# Autodesk Inventor assembly: Assembly1
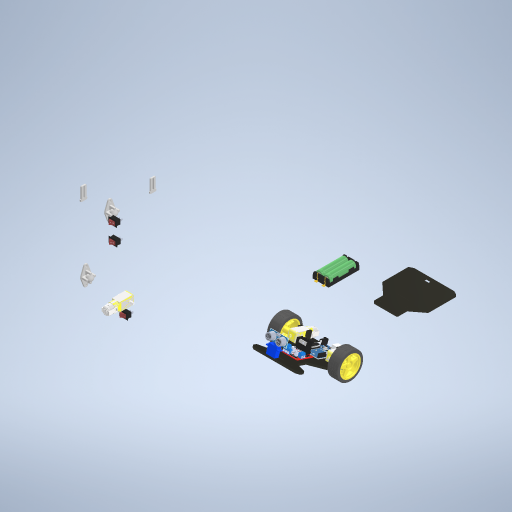
[picture p0: Inventor's stored thumbnail of the model, 512x512]
Saved by Autodesk Inventor 2023 (Build 270158000, 158)
## iProperties
Created: 2023-03-17
Part Number: Assembly1
Document SubType Name: Assembly
Designer: Admins
Author: Admins
## Documents named in this file (15)
- D:\Documents\Researches\Line-Follower-Robot\Assembly1.iam
- D:\Documents\Researches\Line-Follower-Robot\DeTren.ipt
- D:\Documents\Researches\Line-Follower-Robot\KhungDuoi.ipt
- D:\Documents\Researches\Line-Follower-Robot\Parts\Arduino Uno.ipt
- D:\Documents\Researches\Line-Follower-Robot\Parts\Ga motor 1.ipt
- D:\Documents\Researches\Line-Follower-Robot\Parts\HC-SR04.ipt
- D:\Documents\Researches\Line-Follower-Robot\Parts\L298N Stepper Motor Driver (Red).ipt
- D:\Documents\Researches\Line-Follower-Robot\Parts\RockerSwitch.ipt
- D:\Documents\Researches\Line-Follower-Robot\Parts\W420 Ball Caster.ipt
- D:\Documents\Researches\Line-Follower-Robot\Parts\Wheel.ipt
- D:\Documents\Researches\Line-Follower-Robot\Parts\Yellow gear motor.ipt
- D:\Documents\Researches\Line-Follower-Robot\Parts\18650 battery holder.ipt
- D:\Documents\Researches\Line-Follower-Robot\Parts\Yellow gear motor_MIR.ipt
- D:\Documents\Researches\Line-Follower-Robot\Parts\Ga motor 1_MIR.ipt
- D:\Documents\servo-motor-sg90-3.snapshot.3\Servo Motor SG90.ipt
## Components (23 placed, 14 different names)
1. DeTren:1
2. KhungDuoi:1 — Mate:1, Mate:2, Mate:3, Mate:4, Mate:5, Mate:7, Symmetry:1, Mate:12, Flush:1, Mate:15, Flush:2, Mate:17
3. Arduino Uno:1 — Flush:1, Mate:15, Flush:2, Mate:16
4. Ga motor 1:1
5. HC-SR04:1 — Mate:18
6. L298N Stepper Motor Driver (Red):1 — Mate:16
7. RockerSwitch:1
8. W420 Ball Caster:1
9. Wheel:1 — Mate:14
10. Yellow gear motor:1
11. RockerSwitch:2
12. W420 Ball Caster:2
13. Wheel:2 — Mate:13
14. Yellow gear motor:2 — Mate:8, Mate:9, Mate:14
15. 18650 battery holder:1
16. RockerSwitch:3
17. Ga motor 1:2
18. Ga motor 1:3 — Mate:1, Mate:2, Mate:3, Mate:8, Symmetry:1
19. Ga motor 1:4 — Mate:4, Mate:5, Mate:7, Mate:9
20. Yellow gear motor_MIR:1 — Mate:10, Mate:11, Mate:12, Mate:13
21. Ga motor 1_MIR:1 — Mate:10
22. Ga motor 1_MIR:2 — Mate:11
23. Servo Motor SG90:1 — Mate:17, Mate:18
## Relationships (20: Mate 17, Flush 2, Symmetry 1)
- Mate:1: KhungDuoi:1 ↔ Ga motor 1:3
- Mate:2: KhungDuoi:1 ↔ Ga motor 1:3
- Mate:3: KhungDuoi:1 ↔ Ga motor 1:3
- Mate:4: KhungDuoi:1 ↔ Ga motor 1:4
- Mate:5: KhungDuoi:1 ↔ Ga motor 1:4
- Mate:7: KhungDuoi:1 ↔ Ga motor 1:4
- Mate:8: Yellow gear motor:2 ↔ Ga motor 1:3
- Mate:9: Yellow gear motor:2 ↔ Ga motor 1:4
- Symmetry:1: KhungDuoi:1 ↔ Ga motor 1:3
- Mate:10: Yellow gear motor_MIR:1 ↔ Ga motor 1_MIR:1
- Mate:11: Yellow gear motor_MIR:1 ↔ Ga motor 1_MIR:2
- Mate:12: KhungDuoi:1 ↔ Yellow gear motor_MIR:1
- Mate:13: Wheel:2 ↔ Yellow gear motor_MIR:1
- Mate:14: Wheel:1 ↔ Yellow gear motor:2
- Flush:1: KhungDuoi:1 ↔ Arduino Uno:1
- Mate:15: KhungDuoi:1 ↔ Arduino Uno:1
- Flush:2: KhungDuoi:1 ↔ Arduino Uno:1
- Mate:16: Arduino Uno:1 ↔ L298N Stepper Motor Driver (Red):1
- Mate:17: KhungDuoi:1 ↔ Servo Motor SG90:1
- Mate:18: HC-SR04:1 ↔ Servo Motor SG90:1
